# Autodesk Inventor assembly: TCP_verstaerkt
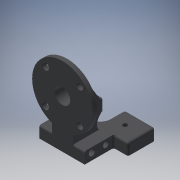
[picture p0: Inventor's stored thumbnail of the model, 180x180]
Saved by Autodesk Inventor 2018 (Build 220112000, 112)
## iProperties
Created: 2018-03-09
Part Number: TCP_verstaerkt
Material: Generisch
Document SubType Name: Assembly
Designer: sebastop
Author: sebastop
## Documents named in this file (3)
- C:\Users\sebas\Documents\Inventor\UR3\TCP_verstaerkt.iam
- C:\Users\sebas\Documents\Inventor\UR3\UR3_Werkzeugaufnahme2.ipt
- C:\Users\sebas\Documents\Inventor\UR3\Extruder_Adapter2.ipt
## Components (2 placed, 2 different names)
1. UR3_Werkzeugaufnahme2:1 — Fluchtend:1, Winkel:1, Passend:1, Passend:2, Passend:3, Passend:4, Passend:5
2. Extruder_Adapter2:1 — Fluchtend:1, Winkel:1, Passend:1, Passend:2
## Relationships (7: Mate 5, Flush 1, Angle 1)
- Fluchtend:1 [Flush]: UR3_Werkzeugaufnahme2:1 ↔ Extruder_Adapter2:1
- Winkel:1 [Angle] (180 deg): UR3_Werkzeugaufnahme2:1 ↔ Extruder_Adapter2:1
- Passend:1 [Mate]: UR3_Werkzeugaufnahme2:1 ↔ Extruder_Adapter2:1
- Passend:2 [Mate]: UR3_Werkzeugaufnahme2:1 ↔ Extruder_Adapter2:1
- Passend:3 [Mate]: UR3_Werkzeugaufnahme2:1
- Passend:4 [Mate]: UR3_Werkzeugaufnahme2:1
- Passend:5 [Mate]: UR3_Werkzeugaufnahme2:1
